# Autodesk Inventor assembly: RPIwCase
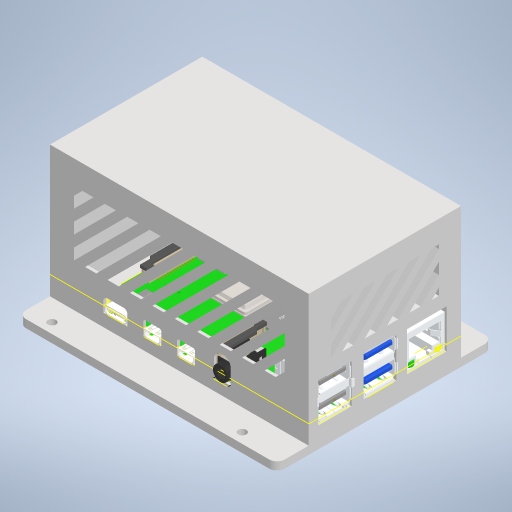
[picture p0: Inventor's stored thumbnail of the model, 512x512]
Saved by Autodesk Inventor 2024 (Build 280153000, 153)
## iProperties
Created: 2023-07-18
Part Number: RPIwCase
Document SubType Name: Assembly
Designer: 18179
Author: 18179
## Documents named in this file (4)
- C:\Users\18179\Desktop\TuppyMkIV\RPIwCase.iam
- C:\Users\18179\Desktop\TuppyMkIV\RPIcaseBottom.ipt
- C:\Users\18179\Desktop\TuppyMkIV\RPI\Raspberry Pi 4 Model B.iam
- C:\Users\18179\Desktop\TuppyMkIV\RPIcaseTop.ipt
## Components (3 placed, 3 different names)
1. RPIcaseBottom:1 — Mate:1, Mate:2, Mate:3, Mate:4, Flush:1, Flush:2
2. Raspberry Pi 4 Model B:1 [sub-assembly] — Mate:1, Mate:2, Mate:3
3. RPIcaseTop:1 — Mate:4, Flush:1, Flush:2
## Relationships (6: Mate 4, Flush 2)
- Mate:1: RPIcaseBottom:1 ↔ Raspberry Pi 4 Model B:1
- Mate:2: RPIcaseBottom:1 ↔ Raspberry Pi 4 Model B:1
- Mate:3: RPIcaseBottom:1 ↔ Raspberry Pi 4 Model B:1
- Mate:4: RPIcaseBottom:1 ↔ RPIcaseTop:1
- Flush:1: RPIcaseBottom:1 ↔ RPIcaseTop:1
- Flush:2: RPIcaseBottom:1 ↔ RPIcaseTop:1
